# Autodesk Inventor assembly: ASY TRM 020 star
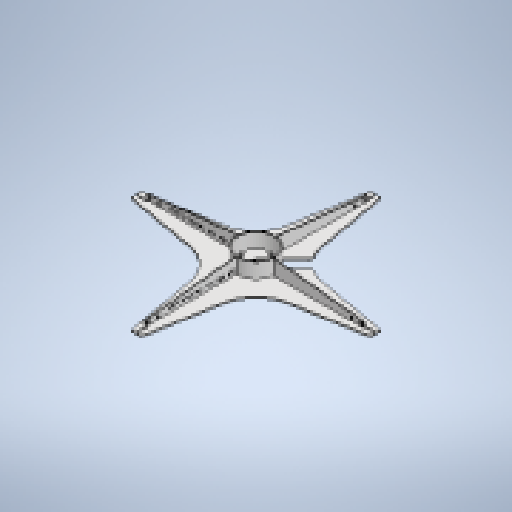
[picture p0: Inventor's stored thumbnail of the model, 512x512]
Saved by Autodesk Inventor 2025.1 (Build 291241020, 241B)
## iProperties
Created: 2024-09-08
Part Number: ASY TRM 020 star
Document SubType Name: Assembly
Designer: pokla
Author: pokla
## Documents named in this file (4)
- C:\Users\user\YandexDisk-badmisterfox\домашниий пк\Inventor\BSH_Beshkino_bio_tank\ASY TRM 020 star.iam
- C:\Users\user\YandexDisk-badmisterfox\домашниий пк\Inventor\BSH_Beshkino_bio_tank\TRM 030 star main.ipt
- C:\Users\user\YandexDisk-badmisterfox\домашниий пк\Inventor\BSH_Beshkino_bio_tank\TRM 032 contrforce ring.ipt
- C:\Users\user\YandexDisk-badmisterfox\домашниий пк\Inventor\BSH_Beshkino_bio_tank\TRM 030 star conrtforce plate.ipt
## Components (6 placed, 3 different names)
1. TRM 030 star main:1 — Rigid:1, Rigid:2, Rigid:3, Rigid:4
2. TRM 032 contrforce ring:1
3. TRM 030 star conrtforce plate:1 — Rigid:1
4. TRM 030 star conrtforce plate:2 — Rigid:2
5. TRM 030 star conrtforce plate:3 — Rigid:3
6. TRM 030 star conrtforce plate:4 — Rigid:4
## Relationships (5: WeldJoint 4, RevoluteJoint 1)
- [RevoluteJoint]: TRM 030 star main:1 ↔ TRM 032 contrforce ring:1
- Rigid:1 [WeldJoint]: TRM 030 star main:1 ↔ TRM 030 star conrtforce plate:1
- Rigid:2 [WeldJoint]: TRM 030 star main:1 ↔ TRM 030 star conrtforce plate:2
- Rigid:3 [WeldJoint]: TRM 030 star main:1 ↔ TRM 030 star conrtforce plate:3
- Rigid:4 [WeldJoint]: TRM 030 star main:1 ↔ TRM 030 star conrtforce plate:4
